# Autodesk Inventor assembly: 全体v1
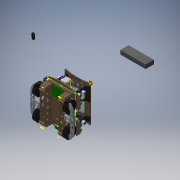
[picture p0: Inventor's stored thumbnail of the model, 180x180]
Saved by Autodesk Inventor 2018.3 (Build 223284000, 284)
## iProperties
Created: 2018-11-27
Part Number: 全体v1
Material: 一般
Document SubType Name: Assembly
Designer: shun2
Author: shun2
## Documents named in this file (21)
- C:\Users\shun2\OneDrive\おそらく最新版(2018.7.31)\全体v1.iam
- C:\Users\shun2\OneDrive\おそらく最新版(2018.7.31)\ギアボックス\ギアボックスv2.iam
- C:\Users\shun2\OneDrive\おそらく最新版(2018.7.31)\1枚目\一枚目.ipt
- C:\Users\shun2\OneDrive\おそらく最新版(2018.7.31)\基板保護2018.8.7.ipt
- C:\Users\shun2\OneDrive\おそらく最新版(2018.7.31)\2枚目\2枚目.ipt
- C:\Users\shun2\OneDrive\おそらく最新版(2018.7.31)\3枚目\3枚目v4.ipt
- C:\Users\shun2\OneDrive\おそらく最新版(2018.7.31)\ping-module.iam
- C:\Users\shun2\OneDrive\おそらく最新版(2018.7.31)\pingmodule-y.iam
- C:\Users\shun2\OneDrive\おそらく最新版(2018.7.31)\OpenMVMount-Tate.iam
- C:\Users\shun2\OneDrive\おそらく最新版(2018.7.31)\Color.ipt
- C:\Users\shun2\OneDrive\おそらく最新版(2018.7.31)\モタドラ.ipt
- C:\Users\shun2\OneDrive\おそらく最新版(2018.7.31)\メイン基板.ipt
- C:\Users\shun2\OneDrive\おそらく最新版(2018.7.31)\Aquila-2018-Under.ipt
- C:\Users\shun2\OneDrive\おそらく最新版(2018.7.31)\LiFePo.ipt
- C:\Users\shun2\OneDrive\おそらく最新版(2018.7.31)\LiFeGuard.ipt
- C:\Users\shun2\OneDrive\おそらく最新版(2018.7.31)\Ping-front.ipt
- C:\Users\shun2\OneDrive\おそらく最新版(2018.7.31)\OpenMVMount-Tate.ipt
- C:\Users\shun2\OneDrive\おそらく最新版(2018.7.31)\microswitch.ipt
- C:\Users\shun2\OneDrive\おそらく最新版(2018.7.31)\Tire.ipt
- C:\Users\shun2\OneDrive\おそらく最新版(2018.7.31)\ガイド\ガイド横v1.ipt
- C:\Users\shun2\OneDrive\おそらく最新版(2018.7.31)\レスキューキット投下機構\RescueKitThrow_Slope.iam
## Components (28 placed, 19 different names)
1. ギアボックスv2:1 [sub-assembly] — メイト:1, フラッシュ:2, フラッシュ:3, メイト:90, メイト:91, メイト:92, メイト:93, メイト:96
2. ギアボックスv2:2 [sub-assembly] — メイト:2, フラッシュ:1, フラッシュ:4, メイト:86, メイト:87, メイト:88, メイト:89
3. 一枚目:1 — メイト:1, メイト:2, フラッシュ:1, フラッシュ:2, フラッシュ:3, フラッシュ:4, メイト:3, メイト:4, メイト:5, メイト:44, メイト:45, メイト:46, メイト:47, メイト:48, メイト:49, メイト:53, メイト:54, メイト:55, メイト:95
4. 基板保護2018.8.7:1 — メイト:3, メイト:4, メイト:5, メイト:6, メイト:7, メイト:8
5. 2枚目:1 — メイト:6, メイト:7, メイト:8, メイト:41, メイト:42, メイト:74, メイト:75, メイト:76, メイト:94, メイト:105, メイト:106, メイト:107, メイト:108, メイト:109, メイト:110, メイト:111, メイト:112, メイト:113, メイト:114, メイト:118, メイト:119
6. 3枚目v4:1 — メイト:29, メイト:30, メイト:31, メイト:41, メイト:42, メイト:50, メイト:51, メイト:52, メイト:58, メイト:59, メイト:60, メイト:64, メイト:65, メイト:66, メイト:80, メイト:94, 回転:1, リジッド:1, メイト:102, メイト:103, メイト:104, メイト:115, メイト:116, メイト:117, メイト:120
7. ping-module:2 [sub-assembly] — メイト:64, メイト:65, メイト:66, メイト:120
8. ping-module:3 [sub-assembly] — メイト:58, メイト:59, メイト:60
9. pingmodule-y:1 [sub-assembly] — メイト:29, メイト:30, メイト:31
10. OpenMVMount-Tate:1 [sub-assembly] — メイト:102, メイト:103
11. OpenMVMount-Tate:2 [sub-assembly] — メイト:80, メイト:104
12. Color:1 — メイト:44, メイト:45, メイト:46
13. モタドラ:1 — メイト:47, メイト:48, メイト:49
14. メイン基板:1 — メイト:50, メイト:51, メイト:52
15. Aquila-2018-Under:2 — メイト:53, メイト:54, メイト:55
16. LiFePo:1
17. LiFeGuard:2 — メイト:108, メイト:109, メイト:110
18. Ping-front:1 — メイト:74, メイト:75, メイト:76
19. OpenMVMount-Tate:3 — 回転:1, リジッド:1
20. microswitch:1
21. Tire:1 — メイト:86, メイト:87
22. Tire:2 — メイト:88, メイト:89
23. Tire:3 — メイト:92, メイト:93
24. Tire:4 — メイト:90, メイト:91
25. ガイド横v1:1 — メイト:105, メイト:106, メイト:107
26. ガイド横v1:2 — メイト:111, メイト:112, メイト:113
27. RescueKitThrow_Slope:1 [sub-assembly] — メイト:114, メイト:118, メイト:119
28. ping-module:4 [sub-assembly] — メイト:115, メイト:116, メイト:117
## Relationships (71: Mate 65, Flush 4, RevoluteJoint 1, WeldJoint 1)
- メイト:1 [Mate] (3 mm): ギアボックスv2:1 ↔ 一枚目:1
- メイト:2 [Mate] (3 mm): ギアボックスv2:2 ↔ 一枚目:1
- フラッシュ:1 [Flush]: ギアボックスv2:2 ↔ 一枚目:1
- フラッシュ:2 [Flush]: ギアボックスv2:1 ↔ 一枚目:1
- フラッシュ:3 [Flush] (2 mm): ギアボックスv2:1 ↔ 一枚目:1
- フラッシュ:4 [Flush] (2 mm): ギアボックスv2:2 ↔ 一枚目:1
- メイト:3 [Mate] (0.2 mm): 一枚目:1 ↔ 基板保護2018.8.7:1
- メイト:4 [Mate]: 一枚目:1 ↔ 基板保護2018.8.7:1
- メイト:5 [Mate]: 一枚目:1 ↔ 基板保護2018.8.7:1
- メイト:6 [Mate] (3 mm): 基板保護2018.8.7:1 ↔ 2枚目:1
- メイト:7 [Mate]: 基板保護2018.8.7:1 ↔ 2枚目:1
- メイト:8 [Mate]: 基板保護2018.8.7:1 ↔ 2枚目:1
- メイト:29 [Mate]: 3枚目v4:1 ↔ pingmodule-y:1
- メイト:30 [Mate]: 3枚目v4:1 ↔ pingmodule-y:1
- メイト:31 [Mate]: 3枚目v4:1 ↔ pingmodule-y:1
- メイト:41 [Mate] (80 mm): 2枚目:1 ↔ 3枚目v4:1
- メイト:42 [Mate]: 2枚目:1 ↔ 3枚目v4:1
- メイト:44 [Mate] (40 mm): 一枚目:1 ↔ Color:1
- メイト:45 [Mate]: 一枚目:1 ↔ Color:1
- メイト:46 [Mate]: 一枚目:1 ↔ Color:1
- メイト:47 [Mate] (8 mm): 一枚目:1 ↔ モタドラ:1
- メイト:48 [Mate]: 一枚目:1 ↔ モタドラ:1
- メイト:49 [Mate]: 一枚目:1 ↔ モタドラ:1
- メイト:50 [Mate] (8 mm): 3枚目v4:1 ↔ メイン基板:1
- メイト:51 [Mate]: 3枚目v4:1 ↔ メイン基板:1
- メイト:52 [Mate]: 3枚目v4:1 ↔ メイン基板:1
- メイト:53 [Mate] (3 mm): 一枚目:1 ↔ Aquila-2018-Under:2
- メイト:54 [Mate]: 一枚目:1 ↔ Aquila-2018-Under:2
- メイト:55 [Mate]: 一枚目:1 ↔ Aquila-2018-Under:2
- メイト:58 [Mate]: 3枚目v4:1 ↔ ping-module:3
- メイト:59 [Mate]: 3枚目v4:1 ↔ ping-module:3
- メイト:60 [Mate]: 3枚目v4:1 ↔ ping-module:3
- メイト:64 [Mate]: 3枚目v4:1 ↔ ping-module:2
- メイト:65 [Mate]: 3枚目v4:1 ↔ ping-module:2
- メイト:66 [Mate]: 3枚目v4:1 ↔ ping-module:2
- メイト:74 [Mate]: 2枚目:1 ↔ Ping-front:1
- メイト:75 [Mate]: 2枚目:1 ↔ Ping-front:1
- メイト:76 [Mate]: 2枚目:1 ↔ Ping-front:1
- メイト:80 [Mate]: 3枚目v4:1 ↔ OpenMVMount-Tate:2
- メイト:86 [Mate] (8 mm): ギアボックスv2:2 ↔ Tire:1
- メイト:87 [Mate]: ギアボックスv2:2 ↔ Tire:1
- メイト:88 [Mate] (8 mm): ギアボックスv2:2 ↔ Tire:2
- メイト:89 [Mate]: ギアボックスv2:2 ↔ Tire:2
- メイト:90 [Mate]: ギアボックスv2:1 ↔ Tire:4
- メイト:91 [Mate] (8 mm): ギアボックスv2:1 ↔ Tire:4
- メイト:92 [Mate]: ギアボックスv2:1 ↔ Tire:3
- メイト:93 [Mate] (8 mm): ギアボックスv2:1 ↔ Tire:3
- メイト:94 [Mate]: 2枚目:1 ↔ 3枚目v4:1
- メイト:95 [Mate]: 一枚目:1
- メイト:96 [Mate]: ギアボックスv2:1
- 回転:1 [RevoluteJoint]: 3枚目v4:1 ↔ OpenMVMount-Tate:3
- リジッド:1 [WeldJoint]: 3枚目v4:1 ↔ OpenMVMount-Tate:3
- メイト:102 [Mate]: 3枚目v4:1 ↔ OpenMVMount-Tate:1
- メイト:103 [Mate]: 3枚目v4:1 ↔ OpenMVMount-Tate:1
- メイト:104 [Mate]: 3枚目v4:1 ↔ OpenMVMount-Tate:2
- メイト:105 [Mate] (45 mm): 2枚目:1 ↔ ガイド横v1:1
- メイト:106 [Mate]: 2枚目:1 ↔ ガイド横v1:1
- メイト:107 [Mate]: 2枚目:1 ↔ ガイド横v1:1
- メイト:108 [Mate]: 2枚目:1 ↔ LiFeGuard:2
- メイト:109 [Mate]: 2枚目:1 ↔ LiFeGuard:2
- メイト:110 [Mate]: 2枚目:1 ↔ LiFeGuard:2
- メイト:111 [Mate] (45 mm): 2枚目:1 ↔ ガイド横v1:2
- メイト:112 [Mate]: 2枚目:1 ↔ ガイド横v1:2
- メイト:113 [Mate]: 2枚目:1 ↔ ガイド横v1:2
- メイト:114 [Mate]: 2枚目:1 ↔ RescueKitThrow_Slope:1
- メイト:115 [Mate]: 3枚目v4:1 ↔ ping-module:4
- メイト:116 [Mate]: 3枚目v4:1 ↔ ping-module:4
- メイト:117 [Mate]: 3枚目v4:1 ↔ ping-module:4
- メイト:118 [Mate]: 2枚目:1 ↔ RescueKitThrow_Slope:1
- メイト:119 [Mate]: 2枚目:1 ↔ RescueKitThrow_Slope:1
- メイト:120 [Mate]: 3枚目v4:1 ↔ ping-module:2
